# Autodesk Inventor assembly: hammerheadeagleIthrust
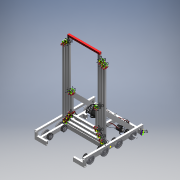
[picture p0: Inventor's stored thumbnail of the model, 180x180]
Saved by Autodesk Inventor 2019 (Build 230136000, 136)
## iProperties
Created: 2019-01-12
Part Number: hammerheadeagleIthrust
Document SubType Name: Assembly
Designer: lebraddock
Mass: 16989.3 g
Surface Area: 41003 cm^2
Volume: 8498.64 cm^3
Density: 1.99906 g/cm^3
Author: lebraddock
## Documents named in this file (21)
- C:\Users\lebraddock\Documents\CameronsRoboticsThings\2019 CAD\hammerheadeagleIthrust.iam
- C:\Users\lebraddock\Documents\CameronsRoboticsThings\2019 CAD\27inchbarchassis.ipt
- C:\Users\lebraddock\Documents\CameronsRoboticsThings\2019 CAD\30inchbarchassis.ipt
- C:\Users\lebraddock\Documents\CameronsRoboticsThings\2019 CAD\13_75mm_1_2_ThunderHex_ID_x_1_125_OD_x_0_313_WD_Flanged_Bearing_217-4006_2.ipt
- C:\Users\lebraddock\Documents\CameronsRoboticsThings\2019 CAD\1.5inch bar.ipt
- C:\Users\lebraddock\Documents\CameronsRoboticsThings\2019 CAD\REV-21-1650.ipt
- C:\Users\lebraddock\Documents\CameronsRoboticsThings\2019 CAD\pullywithhub.iam
- C:\Users\lebraddock\Documents\CameronsRoboticsThings\2019 CAD\Colson_Performa_4_x_0_875_1_2_Hex_bore_217-4049.ipt
- C:\Users\lebraddock\Documents\CameronsRoboticsThings\2019 CAD\1_2_ThunderHex_4Inch.ipt
- C:\Users\lebraddock\Documents\CameronsRoboticsThings\2019 CAD\slider.iam
- C:\Users\lebraddock\Documents\CameronsRoboticsThings\2019 CAD\21inchchassisbar.ipt
- C:\Users\lebraddock\Documents\CameronsRoboticsThings\2019 CAD\18.25x1x1liftbar.ipt
- C:\Users\lebraddock\Documents\CameronsRoboticsThings\2019 CAD\15.5x1x1liftbar.ipt
- C:\Users\lebraddock\Documents\CameronsRoboticsThings\2019 CAD\12.75x1x1liftbar.ipt
- C:\Users\lebraddock\Documents\CameronsRoboticsThings\2019 CAD\liftanglebar.ipt
- C:\Users\lebraddock\Documents\CameronsRoboticsThings\2019 CAD\17.5inch lift bar.ipt
- C:\Users\lebraddock\Documents\CameronsRoboticsThings\2019 CAD\liftCimBar.ipt
- C:\Users\lebraddock\Documents\CameronsRoboticsThings\2019 CAD\WCP_SS_-_WCD_Version_Base_Kit_217-3422.ipt
- C:\Users\lebraddock\Documents\CameronsRoboticsThings\2019 CAD\frontbar6.25.ipt
- C:\Users\lebraddock\Documents\CameronsRoboticsThings\2019 CAD\32inchbumberbar.ipt
- C:\Users\lebraddock\Documents\CameronsRoboticsThings\2019 CAD\1.5inchbar1x1.ipt
## Components (66 placed, 20 different names)
1. 30inchbarchassis:1 — Mate:1, Flush:1, Flush:2, Mate:4, Mate:6, Tangent:7, Tangent:8, Mate:33, Tangent:22, Mate:34, Tangent:23, Mate:66, Flush:17, Flush:18, Mate:68, Flush:19, Flush:20, Mate:73, Flush:34, Mate:80, Mate:81, Mate:82, Mate:83, Tangent:30, Tangent:31, Tangent:34, Tangent:35, Mate:111, Mate:131, Tangent:66, Tangent:67, Mate:138, Flush:53, Flush:54
2. 30inchbarchassis:3 — Mate:2, Flush:3, Flush:4, Mate:8, Mate:10, Tangent:1, Tangent:2, Mate:15, Flush:7, Mate:31, Tangent:20, Mate:32, Tangent:21, Mate:65, Flush:15, Flush:16, Mate:67, Mate:75, Flush:35, Mate:78, Mate:79, Mate:84, Mate:85, Tangent:32, Tangent:36, Tangent:37, Tangent:38, Mate:132, Tangent:68, Tangent:69, Mate:137, Flush:51, Flush:52
3. 27inchbarchassis:1 — Mate:1, Flush:1, Flush:2, Mate:2, Flush:3, Flush:4, Flush:58, Flush:59, Mate:140, Mate:147, Flush:68
4. 13_75mm_1_2_ThunderHex_ID_x_1_125_OD_x_0_313_WD_Flanged_Bearing_217-4006_2:1 — Mate:4, Tangent:8, Flush:12, Tangent:25, Mate:53
5. 13_75mm_1_2_ThunderHex_ID_x_1_125_OD_x_0_313_WD_Flanged_Bearing_217-4006_2:2 — Mate:8, Tangent:2, Flush:14, Tangent:27, Mate:59
6. 13_75mm_1_2_ThunderHex_ID_x_1_125_OD_x_0_313_WD_Flanged_Bearing_217-4006_2:4 — Mate:10, Tangent:1, Mate:47
7. 13_75mm_1_2_ThunderHex_ID_x_1_125_OD_x_0_313_WD_Flanged_Bearing_217-4006_2:6 — Mate:6, Tangent:7, Mate:41
8. 1.5inch bar:1 — Mate:15, Flush:7
9. pullywithhub:4 [sub-assembly]
10. pullywithhub:6 [sub-assembly]
11. Colson_Performa_4_x_0_875_1_2_Hex_bore_217-4049:1 — Mate:38
12. Colson_Performa_4_x_0_875_1_2_Hex_bore_217-4049:2 — Mate:35
13. 13_75mm_1_2_ThunderHex_ID_x_1_125_OD_x_0_313_WD_Flanged_Bearing_217-4006_2:9 — Mate:33, Tangent:22, Mate:38
14. 13_75mm_1_2_ThunderHex_ID_x_1_125_OD_x_0_313_WD_Flanged_Bearing_217-4006_2:10 — Mate:34, Tangent:23
15. 13_75mm_1_2_ThunderHex_ID_x_1_125_OD_x_0_313_WD_Flanged_Bearing_217-4006_2:11 — Mate:31, Tangent:20
16. 13_75mm_1_2_ThunderHex_ID_x_1_125_OD_x_0_313_WD_Flanged_Bearing_217-4006_2:12 — Mate:32, Tangent:21, Mate:35
17. 1_2_ThunderHex_4Inch:1 — Flush:14, Tangent:27, Mate:48, Mate:49, Mate:60, Mate:61
18. 1_2_ThunderHex_4Inch:2 — Flush:12, Tangent:25, Mate:42, Mate:43, Mate:54, Mate:55
19. pullywithhub:7 [sub-assembly] — Mate:47, Mate:48, Mate:49
20. pullywithhub:10 [sub-assembly] — Mate:41, Mate:42, Mate:43
21. Colson_Performa_4_x_0_875_1_2_Hex_bore_217-4049:5 — Mate:59, Mate:60, Mate:61
22. Colson_Performa_4_x_0_875_1_2_Hex_bore_217-4049:6 — Mate:53, Mate:54, Mate:55
23. slider:1 [sub-assembly] — Mate:65, Flush:15, Flush:16, Flush:23, Flush:24, Flush:27, Flush:28, Flush:29, Flush:32, Flush:33, Mate:74, Flush:38, Flush:39
24. slider:2 [sub-assembly] — Mate:66, Flush:17, Flush:18, Mate:69, Flush:21, Flush:22, Mate:70, Flush:25, Flush:26, Mate:71, Flush:30, Flush:31, Mate:72, Mate:76, Flush:36, Flush:37, Mate:77
25. 21inchchassisbar:1 — Mate:67, Mate:68, Flush:19, Flush:20, Mate:110, Flush:44
26. 18.25x1x1liftbar:1 — Mate:69, Flush:21, Flush:22, Flush:23, Flush:24
27. 15.5x1x1liftbar:1 — Mate:70, Flush:25, Flush:26, Flush:27, Flush:28, Flush:29
28. 12.75x1x1liftbar:1 — Mate:71, Flush:30, Flush:31, Flush:32, Flush:33
29. liftanglebar:1 — Mate:74, Mate:75, Flush:35
30. liftanglebar:2 — Mate:72, Mate:73, Flush:34
31. 17.5inch lift bar:1 — Mate:76, Flush:36, Flush:37, Flush:38, Flush:39, Mate:77
32. 13_75mm_1_2_ThunderHex_ID_x_1_125_OD_x_0_313_WD_Flanged_Bearing_217-4006_2:13 — Mate:82, Tangent:30, Flush:41, Tangent:40, Mate:95
33. 13_75mm_1_2_ThunderHex_ID_x_1_125_OD_x_0_313_WD_Flanged_Bearing_217-4006_2:14 — Mate:83, Tangent:31, Flush:40, Tangent:39, Mate:92
34. 13_75mm_1_2_ThunderHex_ID_x_1_125_OD_x_0_313_WD_Flanged_Bearing_217-4006_2:15 — Mate:79, Tangent:37, Flush:42, Tangent:41, Mate:86
35. 13_75mm_1_2_ThunderHex_ID_x_1_125_OD_x_0_313_WD_Flanged_Bearing_217-4006_2:16 — Mate:78, Tangent:36, Flush:43, Tangent:42, Mate:90
36. 13_75mm_1_2_ThunderHex_ID_x_1_125_OD_x_0_313_WD_Flanged_Bearing_217-4006_2:17 — Mate:85, Tangent:38, Mate:98
37. 13_75mm_1_2_ThunderHex_ID_x_1_125_OD_x_0_313_WD_Flanged_Bearing_217-4006_2:18 — Mate:84, Tangent:32, Mate:107
38. 13_75mm_1_2_ThunderHex_ID_x_1_125_OD_x_0_313_WD_Flanged_Bearing_217-4006_2:19 — Mate:81, Tangent:35, Mate:101
39. 13_75mm_1_2_ThunderHex_ID_x_1_125_OD_x_0_313_WD_Flanged_Bearing_217-4006_2:20 — Mate:80, Tangent:34, Mate:104
40. Colson_Performa_4_x_0_875_1_2_Hex_bore_217-4049:7 — Mate:90, Mate:89, Mate:91
41. Colson_Performa_4_x_0_875_1_2_Hex_bore_217-4049:8 — Mate:92, Mate:93, Mate:94
42. Colson_Performa_4_x_0_875_1_2_Hex_bore_217-4049:9 — Mate:86, Mate:87, Mate:88
43. Colson_Performa_4_x_0_875_1_2_Hex_bore_217-4049:10 — Mate:95, Mate:96, Mate:97
44. pullywithhub:11 [sub-assembly] — Mate:101, Mate:102, Mate:103
45. pullywithhub:12 [sub-assembly] — Mate:98, Mate:99, Mate:100
46. pullywithhub:13 [sub-assembly] — Mate:104, Mate:105, Mate:106
47. pullywithhub:14 [sub-assembly] — Mate:107, Mate:108, Mate:109
48. 1_2_ThunderHex_4Inch:3 — Flush:41, Tangent:40, Mate:96, Mate:97, Mate:105, Mate:106
49. 1_2_ThunderHex_4Inch:4 — Flush:43, Tangent:42, Mate:89, Mate:91, Mate:108, Mate:109
50. 1_2_ThunderHex_4Inch:5 — Flush:42, Tangent:41, Mate:87, Mate:88, Mate:99, Mate:100
51. 1_2_ThunderHex_4Inch:6 — Flush:40, Tangent:39, Mate:93, Mate:94, Mate:102, Mate:103
52. liftCimBar:1 — Mate:110, Flush:44, Mate:111
53. WCP_SS_-_WCD_Version_Base_Kit_217-3422:1 — Mate:127, Tangent:58, Tangent:59, Mate:128, Tangent:64, Tangent:65, Mate:131, Tangent:66, Tangent:67
54. WCP_SS_-_WCD_Version_Base_Kit_217-3422:2 — Tangent:60, Tangent:61, Mate:129, Mate:130, Tangent:62, Tangent:63, Mate:132, Tangent:68, Tangent:69
55. REV-21-1650:1 — Tangent:60, Tangent:61, Mate:129
56. REV-21-1650:2 — Mate:130, Tangent:62, Tangent:63
57. REV-21-1650:3 — Tangent:58, Tangent:59, Mate:128
58. REV-21-1650:4 — Mate:127, Tangent:64, Tangent:65
59. frontbar6.25:1 — Mate:137, Flush:51, Flush:52, Mate:139, Flush:55, Flush:56
60. frontbar6.25:2 — Mate:138, Flush:53, Flush:54, Mate:145, Flush:64, Flush:65
61. 32inchbumberbar:2 — Mate:141, Flush:60, Mate:142, Flush:61
62. 1.5inchbar1x1:1 — Flush:58, Flush:59, Mate:140, Mate:141, Flush:60
63. 1.5inchbar1x1:2 — Mate:139, Flush:55, Flush:56, Mate:142, Flush:61
64. 32inchbumberbar:3 — Mate:146, Flush:66, Flush:67
65. 1.5inchbar1x1:3 — Mate:147, Flush:68
66. 1.5inchbar1x1:4 — Mate:145, Flush:64, Flush:65, Mate:146, Flush:66, Flush:67
## Relationships (177: Mate 89, Flush 54, Tangent 34)
- Mate:1: 30inchbarchassis:1 ↔ 27inchbarchassis:1
- Flush:1: 30inchbarchassis:1 ↔ 27inchbarchassis:1
- Flush:2 (50.8 mm): 30inchbarchassis:1 ↔ 27inchbarchassis:1
- Mate:2: 30inchbarchassis:3 ↔ 27inchbarchassis:1
- Flush:3: 30inchbarchassis:3 ↔ 27inchbarchassis:1
- Flush:4 (50.8 mm): 30inchbarchassis:3 ↔ 27inchbarchassis:1
- Mate:4: 30inchbarchassis:1 ↔ 13_75mm_1_2_ThunderHex_ID_x_1_125_OD_x_0_313_WD_Flanged_Bearing_217-4006_2:1
- Mate:6: 30inchbarchassis:1 ↔ 13_75mm_1_2_ThunderHex_ID_x_1_125_OD_x_0_313_WD_Flanged_Bearing_217-4006_2:6
- Mate:8: 30inchbarchassis:3 ↔ 13_75mm_1_2_ThunderHex_ID_x_1_125_OD_x_0_313_WD_Flanged_Bearing_217-4006_2:2
- Mate:10: 30inchbarchassis:3 ↔ 13_75mm_1_2_ThunderHex_ID_x_1_125_OD_x_0_313_WD_Flanged_Bearing_217-4006_2:4
- Tangent:1: 30inchbarchassis:3 ↔ 13_75mm_1_2_ThunderHex_ID_x_1_125_OD_x_0_313_WD_Flanged_Bearing_217-4006_2:4
- Tangent:2: 30inchbarchassis:3 ↔ 13_75mm_1_2_ThunderHex_ID_x_1_125_OD_x_0_313_WD_Flanged_Bearing_217-4006_2:2
- Tangent:7: 30inchbarchassis:1 ↔ 13_75mm_1_2_ThunderHex_ID_x_1_125_OD_x_0_313_WD_Flanged_Bearing_217-4006_2:6
- Tangent:8: 30inchbarchassis:1 ↔ 13_75mm_1_2_ThunderHex_ID_x_1_125_OD_x_0_313_WD_Flanged_Bearing_217-4006_2:1
- Mate:15: 30inchbarchassis:3 ↔ 1.5inch bar:1
- Flush:7: 30inchbarchassis:3 ↔ 1.5inch bar:1
- Mate:31: 30inchbarchassis:3 ↔ 13_75mm_1_2_ThunderHex_ID_x_1_125_OD_x_0_313_WD_Flanged_Bearing_217-4006_2:11
- Tangent:20: 30inchbarchassis:3 ↔ 13_75mm_1_2_ThunderHex_ID_x_1_125_OD_x_0_313_WD_Flanged_Bearing_217-4006_2:11
- Mate:32: 30inchbarchassis:3 ↔ 13_75mm_1_2_ThunderHex_ID_x_1_125_OD_x_0_313_WD_Flanged_Bearing_217-4006_2:12
- Tangent:21: 30inchbarchassis:3 ↔ 13_75mm_1_2_ThunderHex_ID_x_1_125_OD_x_0_313_WD_Flanged_Bearing_217-4006_2:12
- Mate:33: 30inchbarchassis:1 ↔ 13_75mm_1_2_ThunderHex_ID_x_1_125_OD_x_0_313_WD_Flanged_Bearing_217-4006_2:9
- Tangent:22: 30inchbarchassis:1 ↔ 13_75mm_1_2_ThunderHex_ID_x_1_125_OD_x_0_313_WD_Flanged_Bearing_217-4006_2:9
- Mate:34: 30inchbarchassis:1 ↔ 13_75mm_1_2_ThunderHex_ID_x_1_125_OD_x_0_313_WD_Flanged_Bearing_217-4006_2:10
- Tangent:23: 30inchbarchassis:1 ↔ 13_75mm_1_2_ThunderHex_ID_x_1_125_OD_x_0_313_WD_Flanged_Bearing_217-4006_2:10
- Mate:35 (3.175 mm): Colson_Performa_4_x_0_875_1_2_Hex_bore_217-4049:2 ↔ 13_75mm_1_2_ThunderHex_ID_x_1_125_OD_x_0_313_WD_Flanged_Bearing_217-4006_2:12
- Mate:38: Colson_Performa_4_x_0_875_1_2_Hex_bore_217-4049:1 ↔ 13_75mm_1_2_ThunderHex_ID_x_1_125_OD_x_0_313_WD_Flanged_Bearing_217-4006_2:9
- Flush:12 (-31.75 mm): 13_75mm_1_2_ThunderHex_ID_x_1_125_OD_x_0_313_WD_Flanged_Bearing_217-4006_2:1 ↔ 1_2_ThunderHex_4Inch:2
- Tangent:25: 13_75mm_1_2_ThunderHex_ID_x_1_125_OD_x_0_313_WD_Flanged_Bearing_217-4006_2:1 ↔ 1_2_ThunderHex_4Inch:2
- Flush:14 (-31.75 mm): 13_75mm_1_2_ThunderHex_ID_x_1_125_OD_x_0_313_WD_Flanged_Bearing_217-4006_2:2 ↔ 1_2_ThunderHex_4Inch:1
- Tangent:27: 13_75mm_1_2_ThunderHex_ID_x_1_125_OD_x_0_313_WD_Flanged_Bearing_217-4006_2:2 ↔ 1_2_ThunderHex_4Inch:1
- Mate:41 (3.175 mm): 13_75mm_1_2_ThunderHex_ID_x_1_125_OD_x_0_313_WD_Flanged_Bearing_217-4006_2:6 ↔ pullywithhub:10
- Mate:42: 1_2_ThunderHex_4Inch:2 ↔ pullywithhub:10
- Mate:43: 1_2_ThunderHex_4Inch:2 ↔ pullywithhub:10
- Mate:47 (3.175 mm): 13_75mm_1_2_ThunderHex_ID_x_1_125_OD_x_0_313_WD_Flanged_Bearing_217-4006_2:4 ↔ pullywithhub:7
- Mate:48: 1_2_ThunderHex_4Inch:1 ↔ pullywithhub:7
- Mate:49: 1_2_ThunderHex_4Inch:1 ↔ pullywithhub:7
- Mate:53 (3.175 mm): 13_75mm_1_2_ThunderHex_ID_x_1_125_OD_x_0_313_WD_Flanged_Bearing_217-4006_2:1 ↔ Colson_Performa_4_x_0_875_1_2_Hex_bore_217-4049:6
- Mate:54: 1_2_ThunderHex_4Inch:2 ↔ Colson_Performa_4_x_0_875_1_2_Hex_bore_217-4049:6
- Mate:55: 1_2_ThunderHex_4Inch:2 ↔ Colson_Performa_4_x_0_875_1_2_Hex_bore_217-4049:6
- Mate:59 (3.175 mm): 13_75mm_1_2_ThunderHex_ID_x_1_125_OD_x_0_313_WD_Flanged_Bearing_217-4006_2:2 ↔ Colson_Performa_4_x_0_875_1_2_Hex_bore_217-4049:5
- Mate:60: 1_2_ThunderHex_4Inch:1 ↔ Colson_Performa_4_x_0_875_1_2_Hex_bore_217-4049:5
- Mate:61: 1_2_ThunderHex_4Inch:1 ↔ Colson_Performa_4_x_0_875_1_2_Hex_bore_217-4049:5
- Mate:65: 30inchbarchassis:3 ↔ slider:1
- Flush:15: 30inchbarchassis:3 ↔ slider:1
- Flush:16 (304.8 mm): 30inchbarchassis:3 ↔ slider:1
- Mate:66: 30inchbarchassis:1 ↔ slider:2
- Flush:17: 30inchbarchassis:1 ↔ slider:2
- Flush:18 (304.8 mm): 30inchbarchassis:1 ↔ slider:2
- Mate:67: 30inchbarchassis:3 ↔ 21inchchassisbar:1
- Mate:68: 30inchbarchassis:1 ↔ 21inchchassisbar:1
- Flush:19: 30inchbarchassis:1 ↔ 21inchchassisbar:1
- Flush:20 (330.2 mm): 30inchbarchassis:1 ↔ 21inchchassisbar:1
- Mate:69: slider:2 ↔ 18.25x1x1liftbar:1
- Flush:21: slider:2 ↔ 18.25x1x1liftbar:1
- Flush:22: slider:2 ↔ 18.25x1x1liftbar:1
- Flush:23: slider:1 ↔ 18.25x1x1liftbar:1
- Flush:24: slider:1 ↔ 18.25x1x1liftbar:1
- Mate:70: slider:2 ↔ 15.5x1x1liftbar:1
- Flush:25: slider:2 ↔ 15.5x1x1liftbar:1
- Flush:26: slider:2 ↔ 15.5x1x1liftbar:1
- Flush:27: slider:1 ↔ 15.5x1x1liftbar:1
- Flush:28: slider:1 ↔ 15.5x1x1liftbar:1
- Flush:29: slider:1 ↔ 15.5x1x1liftbar:1
- Mate:71: slider:2 ↔ 12.75x1x1liftbar:1
- Flush:30: slider:2 ↔ 12.75x1x1liftbar:1
- Flush:31: slider:2 ↔ 12.75x1x1liftbar:1
- Flush:32: slider:1 ↔ 12.75x1x1liftbar:1
- Flush:33: slider:1 ↔ 12.75x1x1liftbar:1
- Mate:72: slider:2 ↔ liftanglebar:2
- Mate:73: 30inchbarchassis:1 ↔ liftanglebar:2
- Flush:34: 30inchbarchassis:1 ↔ liftanglebar:2
- Mate:74: slider:1 ↔ liftanglebar:1
- Mate:75: 30inchbarchassis:3 ↔ liftanglebar:1
- Flush:35: 30inchbarchassis:3 ↔ liftanglebar:1
- Mate:76: slider:2 ↔ 17.5inch lift bar:1
- Flush:36: slider:2 ↔ 17.5inch lift bar:1
- Flush:37: slider:2 ↔ 17.5inch lift bar:1
- Flush:38: slider:1 ↔ 17.5inch lift bar:1
- Flush:39: slider:1 ↔ 17.5inch lift bar:1
- Mate:77: slider:2 ↔ 17.5inch lift bar:1
- Mate:78: 30inchbarchassis:3 ↔ 13_75mm_1_2_ThunderHex_ID_x_1_125_OD_x_0_313_WD_Flanged_Bearing_217-4006_2:16
- Mate:79: 30inchbarchassis:3 ↔ 13_75mm_1_2_ThunderHex_ID_x_1_125_OD_x_0_313_WD_Flanged_Bearing_217-4006_2:15
- Mate:80: 30inchbarchassis:1 ↔ 13_75mm_1_2_ThunderHex_ID_x_1_125_OD_x_0_313_WD_Flanged_Bearing_217-4006_2:20
- Mate:81: 30inchbarchassis:1 ↔ 13_75mm_1_2_ThunderHex_ID_x_1_125_OD_x_0_313_WD_Flanged_Bearing_217-4006_2:19
- Mate:82: 30inchbarchassis:1 ↔ 13_75mm_1_2_ThunderHex_ID_x_1_125_OD_x_0_313_WD_Flanged_Bearing_217-4006_2:13
- Mate:83: 30inchbarchassis:1 ↔ 13_75mm_1_2_ThunderHex_ID_x_1_125_OD_x_0_313_WD_Flanged_Bearing_217-4006_2:14
- Mate:84: 30inchbarchassis:3 ↔ 13_75mm_1_2_ThunderHex_ID_x_1_125_OD_x_0_313_WD_Flanged_Bearing_217-4006_2:18
- Mate:85: 30inchbarchassis:3 ↔ 13_75mm_1_2_ThunderHex_ID_x_1_125_OD_x_0_313_WD_Flanged_Bearing_217-4006_2:17
- Tangent:30: 30inchbarchassis:1 ↔ 13_75mm_1_2_ThunderHex_ID_x_1_125_OD_x_0_313_WD_Flanged_Bearing_217-4006_2:13
- Tangent:31: 30inchbarchassis:1 ↔ 13_75mm_1_2_ThunderHex_ID_x_1_125_OD_x_0_313_WD_Flanged_Bearing_217-4006_2:14
- Tangent:32: 30inchbarchassis:3 ↔ 13_75mm_1_2_ThunderHex_ID_x_1_125_OD_x_0_313_WD_Flanged_Bearing_217-4006_2:18
- Tangent:34: 30inchbarchassis:1 ↔ 13_75mm_1_2_ThunderHex_ID_x_1_125_OD_x_0_313_WD_Flanged_Bearing_217-4006_2:20
- Tangent:35: 30inchbarchassis:1 ↔ 13_75mm_1_2_ThunderHex_ID_x_1_125_OD_x_0_313_WD_Flanged_Bearing_217-4006_2:19
- Tangent:36: 30inchbarchassis:3 ↔ 13_75mm_1_2_ThunderHex_ID_x_1_125_OD_x_0_313_WD_Flanged_Bearing_217-4006_2:16
- Tangent:37: 30inchbarchassis:3 ↔ 13_75mm_1_2_ThunderHex_ID_x_1_125_OD_x_0_313_WD_Flanged_Bearing_217-4006_2:15
- Tangent:38: 30inchbarchassis:3 ↔ 13_75mm_1_2_ThunderHex_ID_x_1_125_OD_x_0_313_WD_Flanged_Bearing_217-4006_2:17
- Flush:40 (-31.75 mm): 13_75mm_1_2_ThunderHex_ID_x_1_125_OD_x_0_313_WD_Flanged_Bearing_217-4006_2:14 ↔ 1_2_ThunderHex_4Inch:6
- Tangent:39: 13_75mm_1_2_ThunderHex_ID_x_1_125_OD_x_0_313_WD_Flanged_Bearing_217-4006_2:14 ↔ 1_2_ThunderHex_4Inch:6
- Flush:41 (-31.75 mm): 13_75mm_1_2_ThunderHex_ID_x_1_125_OD_x_0_313_WD_Flanged_Bearing_217-4006_2:13 ↔ 1_2_ThunderHex_4Inch:3
- Tangent:40: 13_75mm_1_2_ThunderHex_ID_x_1_125_OD_x_0_313_WD_Flanged_Bearing_217-4006_2:13 ↔ 1_2_ThunderHex_4Inch:3
- Flush:42 (-31.75 mm): 13_75mm_1_2_ThunderHex_ID_x_1_125_OD_x_0_313_WD_Flanged_Bearing_217-4006_2:15 ↔ 1_2_ThunderHex_4Inch:5
- Tangent:41: 13_75mm_1_2_ThunderHex_ID_x_1_125_OD_x_0_313_WD_Flanged_Bearing_217-4006_2:15 ↔ 1_2_ThunderHex_4Inch:5
- Flush:43 (-31.75 mm): 13_75mm_1_2_ThunderHex_ID_x_1_125_OD_x_0_313_WD_Flanged_Bearing_217-4006_2:16 ↔ 1_2_ThunderHex_4Inch:4
- Tangent:42: 13_75mm_1_2_ThunderHex_ID_x_1_125_OD_x_0_313_WD_Flanged_Bearing_217-4006_2:16 ↔ 1_2_ThunderHex_4Inch:4
- Mate:86 (3.175 mm): 13_75mm_1_2_ThunderHex_ID_x_1_125_OD_x_0_313_WD_Flanged_Bearing_217-4006_2:15 ↔ Colson_Performa_4_x_0_875_1_2_Hex_bore_217-4049:9
- Mate:87: Colson_Performa_4_x_0_875_1_2_Hex_bore_217-4049:9 ↔ 1_2_ThunderHex_4Inch:5
- Mate:88: Colson_Performa_4_x_0_875_1_2_Hex_bore_217-4049:9 ↔ 1_2_ThunderHex_4Inch:5
- Mate:90 (3.175 mm): 13_75mm_1_2_ThunderHex_ID_x_1_125_OD_x_0_313_WD_Flanged_Bearing_217-4006_2:16 ↔ Colson_Performa_4_x_0_875_1_2_Hex_bore_217-4049:7
- Mate:89: Colson_Performa_4_x_0_875_1_2_Hex_bore_217-4049:7 ↔ 1_2_ThunderHex_4Inch:4
- Mate:91: Colson_Performa_4_x_0_875_1_2_Hex_bore_217-4049:7 ↔ 1_2_ThunderHex_4Inch:4
- Mate:92 (3.175 mm): 13_75mm_1_2_ThunderHex_ID_x_1_125_OD_x_0_313_WD_Flanged_Bearing_217-4006_2:14 ↔ Colson_Performa_4_x_0_875_1_2_Hex_bore_217-4049:8
- Mate:93: Colson_Performa_4_x_0_875_1_2_Hex_bore_217-4049:8 ↔ 1_2_ThunderHex_4Inch:6
- Mate:94: Colson_Performa_4_x_0_875_1_2_Hex_bore_217-4049:8 ↔ 1_2_ThunderHex_4Inch:6
- Mate:95 (3.175 mm): 13_75mm_1_2_ThunderHex_ID_x_1_125_OD_x_0_313_WD_Flanged_Bearing_217-4006_2:13 ↔ Colson_Performa_4_x_0_875_1_2_Hex_bore_217-4049:10
- Mate:96: Colson_Performa_4_x_0_875_1_2_Hex_bore_217-4049:10 ↔ 1_2_ThunderHex_4Inch:3
- Mate:97: Colson_Performa_4_x_0_875_1_2_Hex_bore_217-4049:10 ↔ 1_2_ThunderHex_4Inch:3
- Mate:98 (3.175 mm): 13_75mm_1_2_ThunderHex_ID_x_1_125_OD_x_0_313_WD_Flanged_Bearing_217-4006_2:17 ↔ pullywithhub:12
- Mate:99: pullywithhub:12 ↔ 1_2_ThunderHex_4Inch:5
- Mate:100: pullywithhub:12 ↔ 1_2_ThunderHex_4Inch:5
- Mate:101 (3.175 mm): 13_75mm_1_2_ThunderHex_ID_x_1_125_OD_x_0_313_WD_Flanged_Bearing_217-4006_2:19 ↔ pullywithhub:11
- Mate:102: pullywithhub:11 ↔ 1_2_ThunderHex_4Inch:6
- Mate:103: pullywithhub:11 ↔ 1_2_ThunderHex_4Inch:6
- Mate:104: 13_75mm_1_2_ThunderHex_ID_x_1_125_OD_x_0_313_WD_Flanged_Bearing_217-4006_2:20 ↔ pullywithhub:13
- Mate:105: pullywithhub:13 ↔ 1_2_ThunderHex_4Inch:3
- Mate:106: pullywithhub:13 ↔ 1_2_ThunderHex_4Inch:3
- Mate:107 (3.175 mm): 13_75mm_1_2_ThunderHex_ID_x_1_125_OD_x_0_313_WD_Flanged_Bearing_217-4006_2:18 ↔ pullywithhub:14
- Mate:108: pullywithhub:14 ↔ 1_2_ThunderHex_4Inch:4
- Mate:109: pullywithhub:14 ↔ 1_2_ThunderHex_4Inch:4
- Mate:110: 21inchchassisbar:1 ↔ liftCimBar:1
- Flush:44: 21inchchassisbar:1 ↔ liftCimBar:1
- Mate:111 (254 mm): 30inchbarchassis:1 ↔ liftCimBar:1
- Mate:127: WCP_SS_-_WCD_Version_Base_Kit_217-3422:1 ↔ REV-21-1650:4
- Tangent:58: WCP_SS_-_WCD_Version_Base_Kit_217-3422:1 ↔ REV-21-1650:3
- Tangent:59: WCP_SS_-_WCD_Version_Base_Kit_217-3422:1 ↔ REV-21-1650:3
- Mate:128: WCP_SS_-_WCD_Version_Base_Kit_217-3422:1 ↔ REV-21-1650:3
- Tangent:60: WCP_SS_-_WCD_Version_Base_Kit_217-3422:2 ↔ REV-21-1650:1
- Tangent:61: WCP_SS_-_WCD_Version_Base_Kit_217-3422:2 ↔ REV-21-1650:1
- Mate:129: WCP_SS_-_WCD_Version_Base_Kit_217-3422:2 ↔ REV-21-1650:1
- Mate:130: WCP_SS_-_WCD_Version_Base_Kit_217-3422:2 ↔ REV-21-1650:2
- Tangent:62: WCP_SS_-_WCD_Version_Base_Kit_217-3422:2 ↔ REV-21-1650:2
- Tangent:63: WCP_SS_-_WCD_Version_Base_Kit_217-3422:2 ↔ REV-21-1650:2
- Tangent:64: WCP_SS_-_WCD_Version_Base_Kit_217-3422:1 ↔ REV-21-1650:4
- Tangent:65: WCP_SS_-_WCD_Version_Base_Kit_217-3422:1 ↔ REV-21-1650:4
- Mate:131: 30inchbarchassis:1 ↔ WCP_SS_-_WCD_Version_Base_Kit_217-3422:1
- Tangent:66: 30inchbarchassis:1 ↔ WCP_SS_-_WCD_Version_Base_Kit_217-3422:1
- Tangent:67: 30inchbarchassis:1 ↔ WCP_SS_-_WCD_Version_Base_Kit_217-3422:1
- Mate:132: 30inchbarchassis:3 ↔ WCP_SS_-_WCD_Version_Base_Kit_217-3422:2
- Tangent:68: 30inchbarchassis:3 ↔ WCP_SS_-_WCD_Version_Base_Kit_217-3422:2
- Tangent:69: 30inchbarchassis:3 ↔ WCP_SS_-_WCD_Version_Base_Kit_217-3422:2
- Mate:137: 30inchbarchassis:3 ↔ frontbar6.25:1
- Flush:51: 30inchbarchassis:3 ↔ frontbar6.25:1
- Flush:52 (-50.8 mm): 30inchbarchassis:3 ↔ frontbar6.25:1
- Mate:138: 30inchbarchassis:1 ↔ frontbar6.25:2
- Flush:53: 30inchbarchassis:1 ↔ frontbar6.25:2
- Flush:54 (-50.8 mm): 30inchbarchassis:1 ↔ frontbar6.25:2
- Mate:139: frontbar6.25:1 ↔ 1.5inchbar1x1:2
- Flush:55: frontbar6.25:1 ↔ 1.5inchbar1x1:2
- Flush:56: frontbar6.25:1 ↔ 1.5inchbar1x1:2
- Flush:58: 27inchbarchassis:1 ↔ 1.5inchbar1x1:1
- Flush:59: 27inchbarchassis:1 ↔ 1.5inchbar1x1:1
- Mate:140: 27inchbarchassis:1 ↔ 1.5inchbar1x1:1
- Mate:141: 32inchbumberbar:2 ↔ 1.5inchbar1x1:1
- Flush:60: 32inchbumberbar:2 ↔ 1.5inchbar1x1:1
- Mate:142: 32inchbumberbar:2 ↔ 1.5inchbar1x1:2
- Flush:61: 32inchbumberbar:2 ↔ 1.5inchbar1x1:2
- [Mate]: 32inchbumberbar:3 ↔ 1.5inchbar1x1:3
- [Flush]: 32inchbumberbar:3 ↔ 1.5inchbar1x1:3
- [Mate]: 32inchbumberbar:3 ↔ 1.5inchbar1x1:4
- [Flush]: 32inchbumberbar:3 ↔ 1.5inchbar1x1:4
- Mate:145: frontbar6.25:2 ↔ 1.5inchbar1x1:4
- Flush:64: frontbar6.25:2 ↔ 1.5inchbar1x1:4
- Flush:65: frontbar6.25:2 ↔ 1.5inchbar1x1:4
- Mate:146: 32inchbumberbar:3 ↔ 1.5inchbar1x1:4
- Flush:66: 32inchbumberbar:3 ↔ 1.5inchbar1x1:4
- Flush:67: 32inchbumberbar:3 ↔ 1.5inchbar1x1:4
- Mate:147: 27inchbarchassis:1 ↔ 1.5inchbar1x1:3
- Flush:68: 27inchbarchassis:1 ↔ 1.5inchbar1x1:3
## Named parameters: d374_d370 = 0 mm, d375_d371 = 0 mm, d376_d372 = 0 mm, d377_d373 = 0 mm
